# Autodesk Inventor assembly: modelo 2
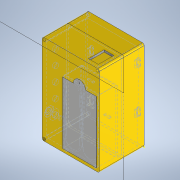
[picture p0: Inventor's stored thumbnail of the model, 180x180]
Saved by Autodesk Inventor 2020 (Build 240168000, 168)
## iProperties
Created: 2022-05-31
Part Number: modelo 2
Document SubType Name: Assembly
Designer: juanc
Author: juanc
## Documents named in this file (5)
- C:\Users\juanc\Desktop\ProyectoIntegrador\3D Model\modelo 2.iam
- C:\Users\juanc\Desktop\ProyectoIntegrador\3D Model\SUPERIOR MODEL2.ipt
- C:\Users\juanc\Desktop\ProyectoIntegrador\3D Model\inferior model2.ipt
- C:\Users\juanc\Desktop\ProyectoIntegrador\3D Model\tapa pila.ipt
- C:\Users\juanc\Desktop\ProyectoIntegrador\3D Model\Banana Hembra.ipt
## Components (4 placed, 4 different names)
1. SUPERIOR MODEL2:1 — Rotational:1
2. inferior model2:1 — Rotational:1, Mate:1, Rotational:2
3. tapa pila:1 — Mate:1
4. Banana Hembra:1 — Rotational:2
## Relationships (3: RevoluteJoint 2, Mate 1)
- Rotational:1 [RevoluteJoint]: SUPERIOR MODEL2:1 ↔ inferior model2:1
- Mate:1: inferior model2:1 ↔ tapa pila:1
- Rotational:2 [RevoluteJoint]: inferior model2:1 ↔ Banana Hembra:1
